# Autodesk Inventor assembly: JHeadmkV
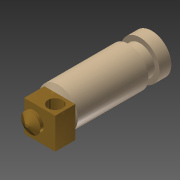
[picture p0: Inventor's stored thumbnail of the model, 180x180]
Saved by Autodesk Inventor 2015 (Build 190159000, 159)
## iProperties
Created: 2014-08-19
Part Number: JHeadmkV
Document SubType Name: Assembly
Designer: t_clevj
Author: t_clevj
## Documents named in this file (3)
- C:\Users\t_clevj\ownCloud\CoreXY\InventorModel\Extruder\JHeadmkV\JHeadmkV.iam
- C:\Users\t_clevj\ownCloud\CoreXY\InventorModel\Extruder\JHeadmkV\JHeadNozzle.ipt
- C:\Users\t_clevj\ownCloud\CoreXY\InventorModel\Extruder\JHeadmkV\JHeadNozzleHolder.ipt
## Components (2 placed, 2 different names)
1. JHeadNozzle:1 — Mate:1, Mate:2
2. JHeadNozzleHolder:1 — Mate:1, Mate:2
## Relationships (2: Mate 2)
- Mate:1: JHeadNozzle:1 ↔ JHeadNozzleHolder:1
- Mate:2: JHeadNozzle:1 ↔ JHeadNozzleHolder:1
